# Autodesk Inventor assembly: Ceiling
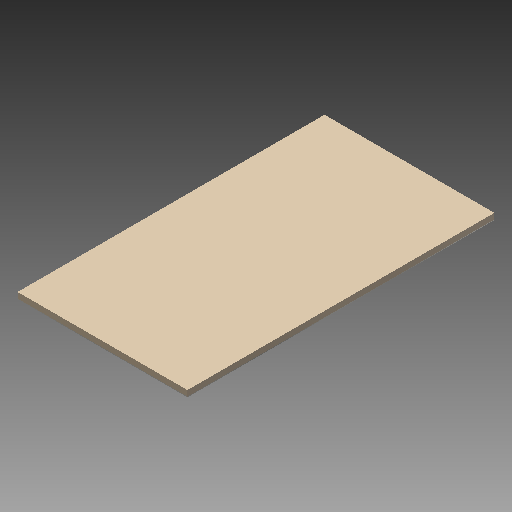
[picture p0: Inventor's stored thumbnail of the model, 512x512]
Saved by Autodesk Inventor 2017 (Build 210142000, 142)
## iProperties
Created: 2016-12-13
Part Number: Ceiling
Document SubType Name: Assembly
Designer: umr
Author: umr
## Documents named in this file (3)
- D:\SeniorProject\Models2\Case\Ceiling.iam
- D:\SeniorProject\Models2\Case\InsulatorCeiling.ipt
- D:\SeniorProject\Models2\Case\ReflectorCeiling.ipt
## Components (2 placed, 2 different names)
1. InsulatorCeiling:1 — Mate:1, Flush:1, Flush:2
2. ReflectorCeiling:1 — Mate:1, Flush:1, Flush:2
## Relationships (3: Flush 2, Mate 1)
- Mate:1: InsulatorCeiling:1 ↔ ReflectorCeiling:1
- Flush:1: InsulatorCeiling:1 ↔ ReflectorCeiling:1
- Flush:2: InsulatorCeiling:1 ↔ ReflectorCeiling:1
